# Autodesk Inventor assembly: wylewanko
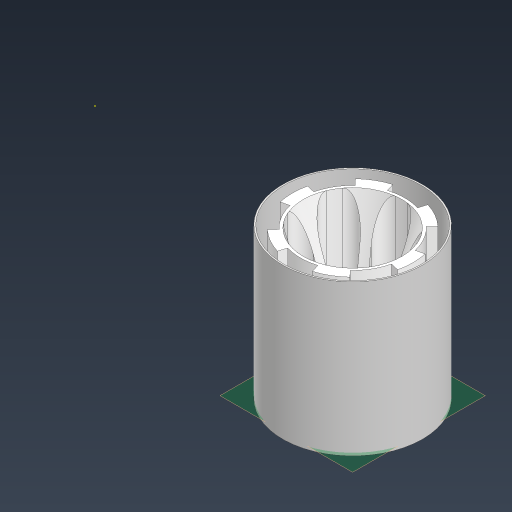
[picture p0: Inventor's stored thumbnail of the model, 512x512]
Saved by Autodesk Inventor 2023 (Build 270158000, 158)
## iProperties
Created: 2025-03-26
Part Number: wylewanko
Document SubType Name: Assembly
Designer: szymo
Author: szymo
## Documents named in this file (3)
- D:\tech\robotyka\robots\codename wafel - australia\3d_parts\rev4\not_in_robot_parts\wylewanko.iam
- D:\tech\robotyka\robots\codename wafel - australia\3d_parts\rev4\felga.ipt
- D:\tech\robotyka\robots\codename wafel - australia\3d_parts\rev4\doWylewanka.ipt
## Components (2 placed, 2 different names)
1. doWylewanka:1 — Flush:3
2. felga:2 — Flush:3
## Relationships (1: Flush 1)
- Flush:3: doWylewanka:1 ↔ felga:2
